# Autodesk Inventor assembly: WormGearExperiment01
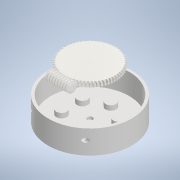
[picture p0: Inventor's stored thumbnail of the model, 180x180]
Saved by Autodesk Inventor 2021 (Build 250183000, 183)
## iProperties
Created: 2020-06-12
Part Number: WormGearExperiment01
Document SubType Name: Assembly
Designer: robst
Author: robst
## Documents named in this file (3)
- C:\git\CAD-Development\robSteele\ShapeWays\TelescopeProjects\TelescopeMount\WormGearExperiment01.iam
- C:\git\CAD-Development\robSteele\ShapeWays\TelescopeProjects\TelescopeMount\baseV01.ipt
- C:\git\CAD-Development\robSteele\ShapeWays\TelescopeProjects\TelescopeMount\WormGearExperiment01\Design Accelerator\Worm Gears1.iam
## Components (2 placed, 2 different names)
1. baseV01:1 — Mate:1, Angle:1
2. Worm Gears:1 [sub-assembly] — Mate:1, Angle:1
## Relationships (2: Mate 1, Angle 1)
- Mate:1: baseV01:1 ↔ Worm Gears:1
- Angle:1 (0 deg): baseV01:1 ↔ Worm Gears:1
